# Autodesk Inventor assembly: GoBilda Viper Slide 4s
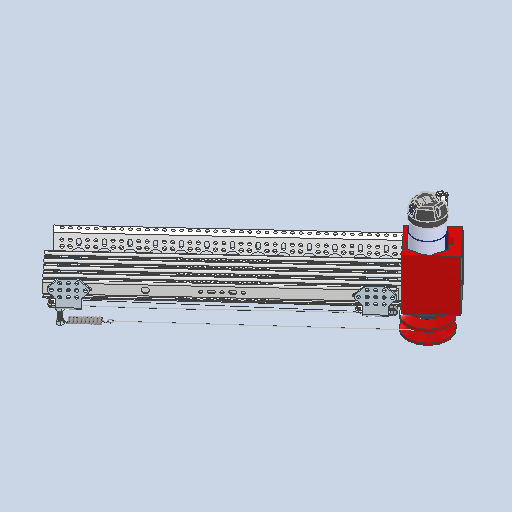
[picture p0: Inventor's stored thumbnail of the model, 512x512]
Saved by Autodesk Inventor 2022 (Build 260153000, 153)
## iProperties
Created: 2022-09-12
Part Number: GoBilda Viper Slide 4s
Description: STEP AP214
Document SubType Name: Assembly
Designer: matt
Preprocessor: ST-DEVELOPER v18.102
Title: 631f7f8adc27ae32af13be63
## Documents named in this file (22)
- C:\Users\matt\Documents\Inventor\FTC\2022-23 FTC\Linear Slide\GoBilda Viper Slide\GoBilda Viper Slide 4s.iam
- C:\Users\matt\Documents\Inventor\FTC\2022-23 FTC\Linear Slide\GoBilda Viper Slide\2501-0001-0001.ipt
- C:\Users\matt\Documents\Inventor\FTC\2022-23 FTC\Linear Slide\GoBilda Viper Slide\1502-0006-0080.ipt
- C:\Users\matt\Documents\Inventor\FTC\2022-23 FTC\Linear Slide\GoBilda Viper Slide\2802-0004-0025.ipt
- C:\Users\matt\Documents\Inventor\FTC\2022-23 FTC\Linear Slide\GoBilda Viper Slide\2802-0004-0005.ipt
- C:\Users\matt\Documents\Inventor\FTC\2022-23 FTC\Linear Slide\GoBilda Viper Slide\2812-0004-0007.ipt
- C:\Users\matt\Documents\Inventor\FTC\2022-23 FTC\Linear Slide\GoBilda Viper Slide\1121-0015-0384.ipt
- C:\Users\matt\Documents\Inventor\FTC\2022-23 FTC\Linear Slide\GoBilda Viper Slide\2802-0004-0014.ipt
- C:\Users\matt\Documents\Inventor\FTC\2022-23 FTC\Linear Slide\GoBilda Viper Slide\2501-0001-0002.ipt
- C:\Users\matt\Documents\Inventor\FTC\2022-23 FTC\Linear Slide\GoBilda Viper Slide\String (RETRACTED) _1_.iam
- C:\Users\matt\Documents\Inventor\FTC\2022-23 FTC\Linear Slide\GoBilda Viper Slide\3408-0001-0001 _2_.iam
- C:\Users\matt\Documents\Inventor\FTC\2022-23 FTC\Linear Slide\GoBilda Viper Slide\2500-0014-0336 _2_.iam
- C:\Users\matt\Documents\Inventor\FTC\2022-23 FTC\Linear Slide\GoBilda Viper Slide\3408-0001-0001 _4_.iam
- C:\Users\matt\Documents\Inventor\FTC\2022-23 FTC\Linear Slide\GoBilda Viper Slide\Assembly 2 _1_.iam
- C:\Users\matt\Documents\Inventor\FTC\2022-23 FTC\Linear Slide\GoBilda Viper Slide\Assembly 2 _3_.iam
- C:\Users\matt\Documents\Inventor\FTC\2022-23 FTC\Linear Slide\GoBilda Viper Slide\3408-0001-0001 _1__2.iam
- C:\Users\matt\Documents\Inventor\FTC\2022-23 FTC\Linear Slide\GoBilda Viper Slide\3408-0001-0001 _3_.iam
- C:\Users\matt\Documents\Inventor\FTC\2022-23 FTC\Linear Slide\GoBilda Viper Slide\2500-0014-0336 _1__2.iam
- C:\Users\matt\Documents\Inventor\FTC\2022-23 FTC\Linear Slide\GoBilda Viper Slide\ViperSlide Motor Mount.ipt
- C:\Users\matt\Documents\Inventor\FTC\2022-23 FTC\Motors\REV Ultraplanetary Motor 2 Cartridges.iam
- C:\Users\matt\Documents\Inventor\FTC\2022-23 FTC\Fasteners\M5 x 25.ipt
- C:\Users\matt\Documents\Inventor\FTC\2022-23 FTC\Linear Slide\GoBilda Viper Slide\Gobilda winch pulley adapter V3.ipt
## Components (43 placed, 43 different names)
1. NAUO1 — Mate:122, Mate:125, Mate:126
2. NAUO2 — Mate:20, Mate:21, Mate:22, Mate:25, Mate:26
3. NAUO5 — Mate:118, Mate:161, Mate:162, Mate:163
4. NAUO9 — Mate:43, Mate:44
5. NAUO10 — Mate:75, Mate:76, Flush:1, Mate:77
6. NAUO15 — Mate:22, Mate:24, Mate:78, Mate:104, Mate:120, Mate:155, Mate:156, Mate:165, Mate:166
7. NAUO16 — Mate:87, Mate:89, Mate:150
8. NAUO17 — Mate:53, Mate:69, Mate:70, Mate:75
9. NAUO18 — Mate:46, Mate:168, Mate:169, Mate:170
10. NAUO30 — Flush:3
11. NAUO31 — Mate:86, Mate:87, Mate:149
12. NAUO39 — Mate:116, Mate:160, Mate:161
13. NAUO40 — Mate:120, Mate:162
14. NAUO41 — Mate:86, Mate:92, Mate:98, Mate:114, Mate:149, Mate:150, Mate:165
15. NAUO42 — Mate:56, Mate:126, Mate:153
16. NAUO43 — Mate:8, Mate:16, Mate:159
17. NAUO48 [sub-assembly] — Mate:18, Mate:19, Mate:28, Mate:29, Mate:38, Mate:39, Mate:40, Mate:41, Mate:42, Mate:50, Mate:52, Mate:53, Mate:54, Mate:55, Mate:140
18. NAUO50 — Mate:1, Mate:2, Mate:3
19. NAUO52 — Mate:48, Mate:168
20. NAUO55 — Mate:20, Mate:27
21. NAUO56 — Mate:89, Mate:92, Mate:145, Mate:148
22. NAUO61 — Mate:58, Mate:59, Mate:125
23. NAUO62 — Mate:69, Mate:70, Mate:71, Mate:72, Mate:76, Mate:83, Mate:112, Mate:113
24. NAUO68 — Mate:71, Mate:72, Mate:77
25. NAUO70 — Mate:4, Mate:5, Mate:6
26. NAUO72 — Mate:172
27. NAUO73 — Mate:8, Mate:9, Mate:43, Mate:44, Mate:46, Mate:48, Mate:167, Mate:169, Mate:171
28. NAUO83 [sub-assembly] — Mate:55, Mate:140, Mate:145, Mate:147, Mate:148
29. NAUO84 — Mate:21, Mate:24
30. NAUO108 [sub-assembly] — Mate:2, Mate:3, Mate:4, Mate:6, Mate:7, Mate:16, Mate:83, Mate:112, Mate:113, Mate:158, Mate:159, Mate:167, Mate:171
31. NAUO109 — Mate:9, Mate:158
32. NAUO118 [sub-assembly] — Mate:50, Mate:116, Mate:118, Mate:163
33. NAUO123 — Mate:57, Mate:58, Mate:59, Mate:121, Mate:122, Mate:141, Mate:142, Mate:154
34. NAUO169 [sub-assembly] — Mate:1, Mate:5, Mate:7, Mate:18, Mate:40, Mate:41, Mate:52, Flush:1, Mate:85
35. NAUO170 — Flush:3, Mate:85
36. NAUO220 [sub-assembly] — Mate:19, Mate:38, Mate:54, Mate:114, Mate:144, Mate:147
37. NAUO229 [sub-assembly] — Mate:25, Mate:26, Mate:27, Mate:28, Mate:29
38. NAUO309 [sub-assembly] — Mate:39, Mate:42, Mate:56, Mate:57, Mate:144, Mate:153, Mate:154
39. NAUO329 [sub-assembly] — Mate:98, Mate:104, Mate:121, Mate:141, Mate:142, Mate:166
40. ViperSlide Motor Mount:1 — Mate:78, Mate:128, Mate:129, Mate:155, Mate:156, Mate:160, Mate:164
41. REV Ultraplanetary Motor 2 Cartridges:1 [sub-assembly] — Mate:128, Mate:129, Mate:164, Mate:173, Mate:174, Mate:175
42. M5 x 25:1 — Mate:170, Mate:172
43. Gobilda winch pulley adapter V3:1 — Mate:173, Mate:174, Mate:175
## Relationships (100: Mate 98, Flush 2)
- Mate:1: NAUO50 ↔ NAUO169
- Mate:2: NAUO50 ↔ NAUO108
- Mate:3: NAUO50 ↔ NAUO108
- Mate:4: NAUO70 ↔ NAUO108
- Mate:5: NAUO70 ↔ NAUO169
- Mate:6: NAUO70 ↔ NAUO108
- Mate:7: NAUO108 ↔ NAUO169
- Mate:8: NAUO43 ↔ NAUO73
- Mate:9: NAUO73 ↔ NAUO109
- Mate:16: NAUO43 ↔ NAUO108
- Mate:18: NAUO48 ↔ NAUO169
- Mate:19: NAUO48 ↔ NAUO220
- Mate:20: NAUO2 ↔ NAUO55
- Mate:21: NAUO2 ↔ NAUO84
- Mate:22: NAUO2 ↔ NAUO15
- Mate:24: NAUO15 ↔ NAUO84
- Mate:25: NAUO2 ↔ NAUO229
- Mate:26: NAUO2 ↔ NAUO229
- Mate:27: NAUO55 ↔ NAUO229
- Mate:28: NAUO48 ↔ NAUO229
- Mate:29 (3.2 mm): NAUO48 ↔ NAUO229
- Mate:38 (3.2 mm): NAUO48 ↔ NAUO220
- Mate:39: NAUO48 ↔ NAUO309
- Mate:40: NAUO48 ↔ NAUO169
- Mate:41 (3.2 mm): NAUO48 ↔ NAUO169
- Mate:42 (3.2 mm): NAUO48 ↔ NAUO309
- Mate:43: NAUO9 ↔ NAUO73
- Mate:44: NAUO9 ↔ NAUO73
- Mate:46: NAUO18 ↔ NAUO73
- Mate:48: NAUO52 ↔ NAUO73
- Mate:50 (3.2 mm): NAUO48 ↔ NAUO118
- Mate:52: NAUO48 ↔ NAUO169
- Mate:53: NAUO17 ↔ NAUO48
- Mate:54: NAUO48 ↔ NAUO220
- Mate:55: NAUO48 ↔ NAUO83
- Mate:56: NAUO42 ↔ NAUO309
- Mate:57: NAUO123 ↔ NAUO309
- Mate:58: NAUO61 ↔ NAUO123
- Mate:59: NAUO61 ↔ NAUO123
- Mate:69: NAUO17 ↔ NAUO62
- Mate:70: NAUO17 ↔ NAUO62
- Mate:71: NAUO62 ↔ NAUO68
- Mate:72: NAUO62 ↔ NAUO68
- Mate:75: NAUO10 ↔ NAUO17
- Mate:76: NAUO10 ↔ NAUO62
- Flush:1: NAUO10 ↔ NAUO169
- Mate:77: NAUO10 ↔ NAUO68
- Mate:78: NAUO15 ↔ ViperSlide Motor Mount:1
- Mate:83: NAUO62 ↔ NAUO108
- Flush:3: NAUO30 ↔ NAUO170
- Mate:85: NAUO169 ↔ NAUO170
- Mate:86: NAUO31 ↔ NAUO41
- Mate:87: NAUO16 ↔ NAUO31
- Mate:89: NAUO16 ↔ NAUO56
- Mate:92: NAUO41 ↔ NAUO56
- Mate:98: NAUO41 ↔ NAUO329
- Mate:104: NAUO15 ↔ NAUO329
- Mate:112: NAUO62 ↔ NAUO108
- Mate:113: NAUO62 ↔ NAUO108
- Mate:114: NAUO41 ↔ NAUO220
- Mate:116: NAUO39 ↔ NAUO118
- Mate:118: NAUO5 ↔ NAUO118
- Mate:120: NAUO15 ↔ NAUO40
- Mate:121: NAUO123 ↔ NAUO329
- Mate:122: NAUO1 ↔ NAUO123
- Mate:125: NAUO1 ↔ NAUO61
- Mate:126: NAUO1 ↔ NAUO42
- Mate:128: ViperSlide Motor Mount:1 ↔ REV Ultraplanetary Motor 2 Cartridges:1
- Mate:129: ViperSlide Motor Mount:1 ↔ REV Ultraplanetary Motor 2 Cartridges:1
- Mate:140: NAUO48 ↔ NAUO83
- Mate:141: NAUO123 ↔ NAUO329
- Mate:142: NAUO123 ↔ NAUO329
- Mate:144: NAUO220 ↔ NAUO309
- Mate:145: NAUO56 ↔ NAUO83
- Mate:147: NAUO83 ↔ NAUO220
- Mate:148: NAUO56 ↔ NAUO83
- Mate:149: NAUO31 ↔ NAUO41
- Mate:150: NAUO16 ↔ NAUO41
- Mate:153: NAUO42 ↔ NAUO309
- Mate:154: NAUO123 ↔ NAUO309
- Mate:155: NAUO15 ↔ ViperSlide Motor Mount:1
- Mate:156: NAUO15 ↔ ViperSlide Motor Mount:1
- Mate:158: NAUO108 ↔ NAUO109
- Mate:159: NAUO43 ↔ NAUO108
- Mate:160: NAUO39 ↔ ViperSlide Motor Mount:1
- Mate:161: NAUO5 ↔ NAUO39
- Mate:162: NAUO5 ↔ NAUO40
- Mate:163: NAUO5 ↔ NAUO118
- Mate:164: ViperSlide Motor Mount:1 ↔ REV Ultraplanetary Motor 2 Cartridges:1
- Mate:165: NAUO15 ↔ NAUO41
- Mate:166: NAUO15 ↔ NAUO329
- Mate:167: NAUO73 ↔ NAUO108
- Mate:168: NAUO18 ↔ NAUO52
- Mate:169: NAUO18 ↔ NAUO73
- Mate:170: NAUO18 ↔ M5 x 25:1
- Mate:171: NAUO73 ↔ NAUO108
- Mate:172: NAUO72 ↔ M5 x 25:1
- Mate:173: REV Ultraplanetary Motor 2 Cartridges:1 ↔ Gobilda winch pulley adapter V3:1
- Mate:174: REV Ultraplanetary Motor 2 Cartridges:1 ↔ Gobilda winch pulley adapter V3:1
- Mate:175: REV Ultraplanetary Motor 2 Cartridges:1 ↔ Gobilda winch pulley adapter V3:1
